# Autodesk Inventor assembly: turns
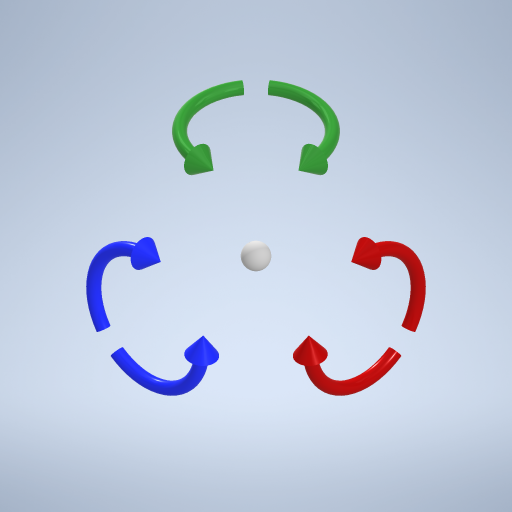
[picture p0: Inventor's stored thumbnail of the model, 512x512]
Saved by Autodesk Inventor 2023 (Build 270158000, 158)
## iProperties
Created: 2022-10-18
Part Number: turns
Document SubType Name: Assembly
Designer: benni
Author: benni
## Documents named in this file (3)
- C:\Users\benni\Documents\GitHub\IR_Assignment2\App Pictures\turns.iam
- C:\Users\benni\Documents\GitHub\IR_Assignment2\App Pictures\Center.ipt
- C:\Users\benni\Documents\GitHub\IR_Assignment2\App Pictures\Turns.ipt
## Components (4 placed, 2 different names)
1. Center:1 — Mate:1
2. Turns:1 — Mate:2, Mate:9, Angle:4
3. Turns:2 — Mate:5, Mate:8, Angle:3
4. Turns:3 — Flush:2, Angle:1, Angle:2, Mate:7
## Relationships (11: Mate 6, Angle 4, Flush 1)
- Mate:1: Center:1
- Mate:2 (20 mm): Turns:1
- Mate:5 (20 mm): Turns:2
- Flush:2 (-20 mm): Turns:3
- Angle:1 (-135 deg): Turns:3
- Angle:2 (135 deg): Turns:3
- Mate:7: Turns:3
- Mate:8: Turns:2
- Angle:3 (45 deg): Turns:2
- Mate:9: Turns:1
- Angle:4 (-135 deg): Turns:1
